# Autodesk Inventor assembly: driveTrain
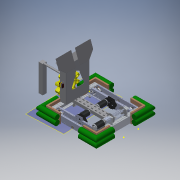
[picture p0: Inventor's stored thumbnail of the model, 180x180]
Saved by Autodesk Inventor 2017 (Build 210142000, 142)
## iProperties
Created: 2017-01-11
Part Number: driveTrain
Document SubType Name: Assembly
Designer: kingb
Author: kingb
## Documents named in this file (26)
- C:\Users\admin\Desktop\CAD\driveTrain.iam
- C:\Users\admin\Desktop\CAD\AM14U3 End Sheet Square.ipt
- C:\Users\admin\Desktop\CAD\AM14U3 Inside Sheet Square.ipt
- C:\Users\admin\Desktop\CAD\AM14U3 Outside Sheet Square.ipt
- C:\Users\admin\Desktop\CAD\10-32 Nylock Nut.ipt
- C:\Users\admin\Desktop\CAD\TM Housing.ipt
- C:\Users\admin\Desktop\CAD\TB Output Shaft Hex L-Base 2.ipt
- C:\Users\admin\Desktop\CAD\FR8ZZ Hex Bearing.ipt
- C:\Users\admin\Desktop\CAD\25inCIM.ipt
- C:\Users\admin\Desktop\CAD\375-16 x 4.25 Hex Bolt_HFBOLT 0.375-16x2.5x1-C.ipt
- C:\Users\admin\Desktop\CAD\375-16 Lock Nut_91831A127.ipt
- C:\Users\admin\Desktop\CAD\customWheelSpacers.ipt
- C:\Users\admin\Desktop\CAD\hookBoi.ipt
- C:\Users\admin\Desktop\CAD\am-3047_4inDuraOmniV2.ipt
- C:\Users\admin\Desktop\CAD\assembledPrototype1.iam
- C:\Users\admin\Desktop\CAD\3230T450_STRUT CHANNEL.ipt
- C:\Users\admin\Desktop\CAD\cameramount.ipt
- C:\Users\admin\Desktop\CAD\Bumper.iam
- C:\Users\admin\Desktop\CAD\cameraMetalExtender.ipt
- C:\Users\admin\Desktop\CAD\lifterB.iam
- C:\Users\admin\Desktop\CAD\MotorCraddle.ipt
- C:\Users\admin\Desktop\CAD\motorMount.ipt
- C:\Users\admin\Desktop\CAD\HSmount.ipt
- C:\Users\admin\Desktop\CAD\HS-322HD.ipt
- C:\Users\admin\Downloads\bearing.ipt
- C:\Users\admin\Downloads\hub.ipt
## Components (55 placed, 25 different names)
1. AM14U3 End Sheet Square:1 — Mate:84, Insert:131, Insert:136, Insert:137, Insert:146, Insert:147, Insert:148, Insert:149, Mate:110, Mate:111, Mate:112, Mate:123, Mate:148, Flush:36, Flush:37, Mate:150, Mate:152, Insert:154, Insert:155, Insert:156, Insert:157, Mate:154
2. AM14U3 Inside Sheet Square:1 — Insert:105, Insert:106, Insert:113, Insert:114, Mate:27, Mate:30, Insert:138, Insert:139, Mate:87, Mate:111
3. AM14U3 Inside Sheet Square:2 — Insert:107, Insert:108, Insert:115, Insert:116, Mate:31, Mate:33, Insert:136, Insert:137, Insert:146, Insert:147
4. AM14U3 Outside Sheet Square:1 — Insert:112, Mate:20, Mate:21, Mate:22, Mate:23, Mate:32, Mate:34, Mate:84, Insert:131, Insert:148, Insert:149, Flush:24, Mate:151
5. AM14U3 Outside Sheet Square:2 — Insert:111, Mate:13, Mate:14, Mate:18, Mate:19, Mate:28, Mate:29, Insert:140, Insert:141, Mate:87, Mate:110, Mate:112, Mate:123, Mate:149, Flush:39
6. AM14U3 End Sheet Square:2 — Flush:1, Angle:3, Insert:127, Insert:128, Insert:129, Insert:130, Mate:82, Insert:138, Insert:139, Insert:140, Insert:141, Mate:86, Flush:23, Mate:145, Angle:11
7. TM Housing:1 — Insert:107, Insert:108, Insert:109, Mate:10, Mate:11, Mate:12
8. TM Housing:2 — Insert:105, Insert:106, Insert:110, Mate:7, Mate:8, Mate:9
9. TB Output Shaft Hex L-Base 2:1 — Insert:109, Angle:2
10. TB Output Shaft Hex L-Base 2:2 — Insert:110, Angle:1
11. FR8ZZ Hex Bearing:1 — Insert:111, Angle:1
12. FR8ZZ Hex Bearing:2 — Insert:112, Angle:2
13. 25inCIM:1 — Mate:10, Mate:11, Mate:12
14. 25inCIM:2 — Mate:7, Mate:8, Mate:9
15. 375-16 x 4.25 Hex Bolt_HFBOLT 0.375-16x2.5x1-C:1 — Mate:22, Mate:23, Mate:37, Mate:38, Mate:64
16. 375-16 x 4.25 Hex Bolt_HFBOLT 0.375-16x2.5x1-C:2 — Mate:20, Mate:21, Mate:35, Mate:36, Mate:65, Angle:7
17. 375-16 x 4.25 Hex Bolt_HFBOLT 0.375-16x2.5x1-C:3 — Mate:13, Mate:14, Mate:41, Mate:42, Mate:62, Angle:9
18. 375-16 x 4.25 Hex Bolt_HFBOLT 0.375-16x2.5x1-C:4 — Mate:18, Mate:19, Mate:39, Mate:40, Mate:63, Angle:8
19. 375-16 Lock Nut_91831A127:1 — Insert:113
20. 375-16 Lock Nut_91831A127:2 — Insert:116
21. 375-16 Lock Nut_91831A127:3 — Insert:114
22. 375-16 Lock Nut_91831A127:4 — Insert:115, Angle:6
23. customWheelSpacers:1 — Mate:28, Mate:40
24. customWheelSpacers:2 — Mate:27, Mate:39
25. customWheelSpacers:3 — Mate:33, Mate:37
26. customWheelSpacers:4 — Mate:34, Mate:38
27. customWheelSpacers:5 — Mate:31, Mate:35
28. customWheelSpacers:6 — Mate:32, Mate:36
29. customWheelSpacers:7 — Mate:29, Mate:41
30. customWheelSpacers:8 — Mate:30, Mate:42
31. hookBoi:1 — Flush:3, Angle:3
32. 10-32 Nylock Nut:41 — Insert:130
33. 10-32 Nylock Nut:42 — Insert:129
34. 10-32 Nylock Nut:43 — Insert:128
35. 10-32 Nylock Nut:44 — Insert:127
36. am-3047_4inDuraOmniV2:1 — Mate:64, Angle:6
37. am-3047_4inDuraOmniV2:2 — Mate:65, Angle:7
38. am-3047_4inDuraOmniV2:3 — Mate:62, Angle:9
39. am-3047_4inDuraOmniV2:4 — Mate:63, Angle:8
40. 3230T450_STRUT CHANNEL:1 — Mate:82, Mate:86, Mate:109, Flush:19, Flush:20
41. 3230T450_STRUT CHANNEL:2 — Mate:109, Flush:19, Flush:20, Flush:39
42. assembledPrototype1:1 [sub-assembly] — Flush:23, Flush:24
43. Bumper:1 [sub-assembly] — Flush:37, Mate:150, Mate:151
44. Bumper:2 [sub-assembly]
45. Bumper:3 [sub-assembly]
46. Bumper:4 [sub-assembly] — Mate:148, Mate:149, Flush:36
47. cameramount:4 — Mate:141, Mate:142, Flush:32, Flush:33, Mate:145, Angle:11
48. cameraMetalExtender:1 — Mate:141, Mate:142, Flush:32, Flush:33
49. lifterB:1 [sub-assembly] — Mate:152, Insert:154, Insert:155, Mate:153
50. MotorCraddle:1 — Insert:156, Insert:157
51. motorMount:1 — Mate:153, Mate:154
52. HSmount:1 — Mate:157, Mate:158, Mate:159, Mate:160
53. HS-322HD:1 — Mate:157, Mate:158, Mate:159, Mate:160
54. bearing:1
55. hub:1
## Relationships (108: Mate 57, Insert 31, Flush 12, Angle 8)
- Insert:105: AM14U3 Inside Sheet Square:1 ↔ TM Housing:2
- Insert:106: AM14U3 Inside Sheet Square:1 ↔ TM Housing:2
- Insert:107: AM14U3 Inside Sheet Square:2 ↔ TM Housing:1
- Insert:108: AM14U3 Inside Sheet Square:2 ↔ TM Housing:1
- Insert:109: TM Housing:1 ↔ TB Output Shaft Hex L-Base 2:1
- Insert:110: TM Housing:2 ↔ TB Output Shaft Hex L-Base 2:2
- Insert:111: AM14U3 Outside Sheet Square:2 ↔ FR8ZZ Hex Bearing:1
- Angle:1 (0 deg): TB Output Shaft Hex L-Base 2:2 ↔ FR8ZZ Hex Bearing:1
- Insert:112: AM14U3 Outside Sheet Square:1 ↔ FR8ZZ Hex Bearing:2
- Angle:2 (0 deg): TB Output Shaft Hex L-Base 2:1 ↔ FR8ZZ Hex Bearing:2
- Mate:7: TM Housing:2 ↔ 25inCIM:2
- Mate:8: TM Housing:2 ↔ 25inCIM:2
- Mate:9: TM Housing:2 ↔ 25inCIM:2
- Mate:10: TM Housing:1 ↔ 25inCIM:1
- Mate:11: TM Housing:1 ↔ 25inCIM:1
- Mate:12: TM Housing:1 ↔ 25inCIM:1
- Mate:13: AM14U3 Outside Sheet Square:2 ↔ 375-16 x 4.25 Hex Bolt_HFBOLT 0.375-16x2.5x1-C:3
- Mate:14: AM14U3 Outside Sheet Square:2 ↔ 375-16 x 4.25 Hex Bolt_HFBOLT 0.375-16x2.5x1-C:3
- Mate:18: AM14U3 Outside Sheet Square:2 ↔ 375-16 x 4.25 Hex Bolt_HFBOLT 0.375-16x2.5x1-C:4
- Mate:19: AM14U3 Outside Sheet Square:2 ↔ 375-16 x 4.25 Hex Bolt_HFBOLT 0.375-16x2.5x1-C:4
- Mate:20: AM14U3 Outside Sheet Square:1 ↔ 375-16 x 4.25 Hex Bolt_HFBOLT 0.375-16x2.5x1-C:2
- Mate:21: AM14U3 Outside Sheet Square:1 ↔ 375-16 x 4.25 Hex Bolt_HFBOLT 0.375-16x2.5x1-C:2
- Mate:22: AM14U3 Outside Sheet Square:1 ↔ 375-16 x 4.25 Hex Bolt_HFBOLT 0.375-16x2.5x1-C:1
- Mate:23: AM14U3 Outside Sheet Square:1 ↔ 375-16 x 4.25 Hex Bolt_HFBOLT 0.375-16x2.5x1-C:1
- Insert:113: AM14U3 Inside Sheet Square:1 ↔ 375-16 Lock Nut_91831A127:1
- Insert:114: AM14U3 Inside Sheet Square:1 ↔ 375-16 Lock Nut_91831A127:3
- Insert:115: AM14U3 Inside Sheet Square:2 ↔ 375-16 Lock Nut_91831A127:4
- Insert:116: AM14U3 Inside Sheet Square:2 ↔ 375-16 Lock Nut_91831A127:2
- Mate:27: AM14U3 Inside Sheet Square:1 ↔ customWheelSpacers:2
- Mate:28: AM14U3 Outside Sheet Square:2 ↔ customWheelSpacers:1
- Mate:29: AM14U3 Outside Sheet Square:2 ↔ customWheelSpacers:7
- Mate:30: AM14U3 Inside Sheet Square:1 ↔ customWheelSpacers:8
- Mate:31: AM14U3 Inside Sheet Square:2 ↔ customWheelSpacers:5
- Mate:32: AM14U3 Outside Sheet Square:1 ↔ customWheelSpacers:6
- Mate:33: AM14U3 Inside Sheet Square:2 ↔ customWheelSpacers:3
- Mate:34: AM14U3 Outside Sheet Square:1 ↔ customWheelSpacers:4
- Mate:35: 375-16 x 4.25 Hex Bolt_HFBOLT 0.375-16x2.5x1-C:2 ↔ customWheelSpacers:5
- Mate:36: 375-16 x 4.25 Hex Bolt_HFBOLT 0.375-16x2.5x1-C:2 ↔ customWheelSpacers:6
- Mate:37: 375-16 x 4.25 Hex Bolt_HFBOLT 0.375-16x2.5x1-C:1 ↔ customWheelSpacers:3
- Mate:38: 375-16 x 4.25 Hex Bolt_HFBOLT 0.375-16x2.5x1-C:1 ↔ customWheelSpacers:4
- Mate:39: 375-16 x 4.25 Hex Bolt_HFBOLT 0.375-16x2.5x1-C:4 ↔ customWheelSpacers:2
- Mate:40: 375-16 x 4.25 Hex Bolt_HFBOLT 0.375-16x2.5x1-C:4 ↔ customWheelSpacers:1
- Mate:41: 375-16 x 4.25 Hex Bolt_HFBOLT 0.375-16x2.5x1-C:3 ↔ customWheelSpacers:7
- Mate:42: 375-16 x 4.25 Hex Bolt_HFBOLT 0.375-16x2.5x1-C:3 ↔ customWheelSpacers:8
- Flush:1 (25.4 mm): AM14U3 End Sheet Square:2
- Flush:2 (-609.6 mm)
- Flush:3: hookBoi:1
- Angle:3 (180 deg): AM14U3 End Sheet Square:2 ↔ hookBoi:1
- Insert:127: AM14U3 End Sheet Square:2 ↔ 10-32 Nylock Nut:44
- Insert:128: AM14U3 End Sheet Square:2 ↔ 10-32 Nylock Nut:43
- Insert:129: AM14U3 End Sheet Square:2 ↔ 10-32 Nylock Nut:42
- Insert:130: AM14U3 End Sheet Square:2 ↔ 10-32 Nylock Nut:41
- Mate:62: 375-16 x 4.25 Hex Bolt_HFBOLT 0.375-16x2.5x1-C:3 ↔ am-3047_4inDuraOmniV2:3
- Mate:63: 375-16 x 4.25 Hex Bolt_HFBOLT 0.375-16x2.5x1-C:4 ↔ am-3047_4inDuraOmniV2:4
- Mate:64: 375-16 x 4.25 Hex Bolt_HFBOLT 0.375-16x2.5x1-C:1 ↔ am-3047_4inDuraOmniV2:1
- Mate:65: 375-16 x 4.25 Hex Bolt_HFBOLT 0.375-16x2.5x1-C:2 ↔ am-3047_4inDuraOmniV2:2
- Angle:6 (0 deg): 375-16 Lock Nut_91831A127:4 ↔ am-3047_4inDuraOmniV2:1
- Angle:7 (0 deg): 375-16 x 4.25 Hex Bolt_HFBOLT 0.375-16x2.5x1-C:2 ↔ am-3047_4inDuraOmniV2:2
- Angle:8 (0 deg): 375-16 x 4.25 Hex Bolt_HFBOLT 0.375-16x2.5x1-C:4 ↔ am-3047_4inDuraOmniV2:4
- Angle:9 (0 deg): 375-16 x 4.25 Hex Bolt_HFBOLT 0.375-16x2.5x1-C:3 ↔ am-3047_4inDuraOmniV2:3
- Mate:82: AM14U3 End Sheet Square:2 ↔ 3230T450_STRUT CHANNEL:1
- Mate:84: AM14U3 End Sheet Square:1 ↔ AM14U3 Outside Sheet Square:1
- Insert:131: AM14U3 End Sheet Square:1 ↔ AM14U3 Outside Sheet Square:1
- Insert:136: AM14U3 End Sheet Square:1 ↔ AM14U3 Inside Sheet Square:2
- Insert:137: AM14U3 End Sheet Square:1 ↔ AM14U3 Inside Sheet Square:2
- Insert:138: AM14U3 Inside Sheet Square:1 ↔ AM14U3 End Sheet Square:2
- Insert:139: AM14U3 Inside Sheet Square:1 ↔ AM14U3 End Sheet Square:2
- Insert:140: AM14U3 Outside Sheet Square:2 ↔ AM14U3 End Sheet Square:2
- Insert:141: AM14U3 Outside Sheet Square:2 ↔ AM14U3 End Sheet Square:2
- Mate:86: AM14U3 End Sheet Square:2 ↔ 3230T450_STRUT CHANNEL:1
- Mate:87 (85.725 mm): AM14U3 Inside Sheet Square:1 ↔ AM14U3 Outside Sheet Square:2
- Insert:146: AM14U3 End Sheet Square:1 ↔ AM14U3 Inside Sheet Square:2
- Insert:147: AM14U3 End Sheet Square:1 ↔ AM14U3 Inside Sheet Square:2
- Insert:148: AM14U3 End Sheet Square:1 ↔ AM14U3 Outside Sheet Square:1
- Insert:149: AM14U3 End Sheet Square:1 ↔ AM14U3 Outside Sheet Square:1
- Mate:109: 3230T450_STRUT CHANNEL:1 ↔ 3230T450_STRUT CHANNEL:2
- Flush:19: 3230T450_STRUT CHANNEL:1 ↔ 3230T450_STRUT CHANNEL:2
- Flush:20: 3230T450_STRUT CHANNEL:1 ↔ 3230T450_STRUT CHANNEL:2
- Mate:110: AM14U3 End Sheet Square:1 ↔ AM14U3 Outside Sheet Square:2
- Mate:111: AM14U3 End Sheet Square:1 ↔ AM14U3 Inside Sheet Square:1
- Mate:112: AM14U3 End Sheet Square:1 ↔ AM14U3 Outside Sheet Square:2
- Flush:23: AM14U3 End Sheet Square:2 ↔ assembledPrototype1:1
- Flush:24 (146.05 mm): AM14U3 Outside Sheet Square:1 ↔ assembledPrototype1:1
- Mate:123: AM14U3 End Sheet Square:1 ↔ AM14U3 Outside Sheet Square:2
- Mate:141: cameramount:4 ↔ cameraMetalExtender:1
- Mate:142: cameramount:4 ↔ cameraMetalExtender:1
- Flush:32: cameramount:4 ↔ cameraMetalExtender:1
- Flush:33: cameramount:4 ↔ cameraMetalExtender:1
- Mate:145: AM14U3 End Sheet Square:2 ↔ cameramount:4
- Angle:11 (-30 deg): AM14U3 End Sheet Square:2 ↔ cameramount:4
- Mate:148: AM14U3 End Sheet Square:1 ↔ Bumper:4
- Mate:149: AM14U3 Outside Sheet Square:2 ↔ Bumper:4
- Flush:36: AM14U3 End Sheet Square:1 ↔ Bumper:4
- Flush:37: AM14U3 End Sheet Square:1 ↔ Bumper:1
- Mate:150: AM14U3 End Sheet Square:1 ↔ Bumper:1
- Mate:151: AM14U3 Outside Sheet Square:1 ↔ Bumper:1
- Flush:39 (257.175 mm): AM14U3 Outside Sheet Square:2 ↔ 3230T450_STRUT CHANNEL:2
- Mate:152: AM14U3 End Sheet Square:1 ↔ lifterB:1
- Insert:154: AM14U3 End Sheet Square:1 ↔ lifterB:1
- Insert:155: AM14U3 End Sheet Square:1 ↔ lifterB:1
- Insert:156: AM14U3 End Sheet Square:1 ↔ MotorCraddle:1
- Insert:157: AM14U3 End Sheet Square:1 ↔ MotorCraddle:1
- Mate:153: lifterB:1 ↔ motorMount:1
- Mate:154: AM14U3 End Sheet Square:1 ↔ motorMount:1
- Mate:157: HSmount:1 ↔ HS-322HD:1
- Mate:158: HSmount:1 ↔ HS-322HD:1
- Mate:159: HSmount:1 ↔ HS-322HD:1
- Mate:160: HSmount:1 ↔ HS-322HD:1
